# Autodesk Inventor assembly: Center Frame SEC
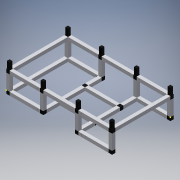
[picture p0: Inventor's stored thumbnail of the model, 180x180]
Saved by Autodesk Inventor 2017 (Build 210142000, 142)
## iProperties
Created: 2019-12-06
Part Number: Center Frame SEC
Document SubType Name: Assembly
Designer: S346553810
Author: S346553810
## Documents named in this file (7)
- \\ad.ocdsb.ca\studenthome\3\S338674153\FRC 2020\FullRobotRefactor\SubFrame\Center Frame SEC.iam
- \\ad.ocdsb.ca\studenthome\3\S338674153\FRC 2020\FullRobotRefactor\SubFrame\Center Assembly.iam
- \\ad.ocdsb.ca\studenthome\3\S338674153\FRC 2020\FullRobotRefactor\SubFrame\Frame End.iam
- \\ad.ocdsb.ca\studenthome\3\S338674153\FRC 2020\FullRobotRefactor\SubFrame\90 joint piece.ipt
- \\ad.ocdsb.ca\studenthome\3\S338674153\FRC 2020\FullRobotRefactor\SubFrame\lower piece.ipt
- \\ad.ocdsb.ca\studenthome\3\S338674153\FRC 2020\FullRobotRefactor\SubFrame\roller hole piece.ipt
- \\ad.ocdsb.ca\studenthome\3\S338674153\FRC 2020\FullRobotRefactor\SubFrame\Kipp K0619.ipt
## Components (12 placed, 6 different names)
1. Center Assembly:1 [sub-assembly] — Flush:33, Flush:34, Flush:35, Mate:36
2. Frame End:1 [sub-assembly] — Mate:29, Mate:30, Mate:31, Flush:26, Flush:27, Mate:34, Flush:28, Flush:29, Mate:35, Flush:30, Flush:32, Flush:33, Flush:34, Flush:35, Mate:36
3. Frame End:2 [sub-assembly] — Mate:33, Flush:22, Flush:23
4. 90 joint piece:1 — Mate:24, Flush:20, Flush:21
5. 90 joint piece:2 — Mate:23, Flush:18, Flush:19, Mate:33, Flush:22
6. lower piece:1 — Flush:24, Flush:25, Flush:31, Mate:37
7. roller hole piece:2 — Mate:23, Flush:18, Flush:19, Flush:23
8. roller hole piece:3 — Mate:24, Flush:20, Flush:21
9. roller hole piece:4 — Mate:29, Mate:30, Mate:31
10. roller hole piece:5 — Flush:28, Flush:29, Mate:35
11. Kipp K0619:1 — Flush:24, Flush:25, Flush:26, Flush:27, Mate:34, Mate:37
12. Kipp K0619:2 — Flush:30, Flush:31, Flush:32
## Relationships (28: Flush 18, Mate 10)
- Mate:23: 90 joint piece:2 ↔ roller hole piece:2
- Flush:18: 90 joint piece:2 ↔ roller hole piece:2
- Flush:19: 90 joint piece:2 ↔ roller hole piece:2
- Mate:24: 90 joint piece:1 ↔ roller hole piece:3
- Flush:20: 90 joint piece:1 ↔ roller hole piece:3
- Flush:21: 90 joint piece:1 ↔ roller hole piece:3
- Mate:29: Frame End:1 ↔ roller hole piece:4
- Mate:30: Frame End:1 ↔ roller hole piece:4
- Mate:31: Frame End:1 ↔ roller hole piece:4
- Mate:33: Frame End:2 ↔ 90 joint piece:2
- Flush:22: Frame End:2 ↔ 90 joint piece:2
- Flush:23: Frame End:2 ↔ roller hole piece:2
- Flush:24: lower piece:1 ↔ Kipp K0619:1
- Flush:25: lower piece:1 ↔ Kipp K0619:1
- Flush:26: Frame End:1 ↔ Kipp K0619:1
- Flush:27: Frame End:1 ↔ Kipp K0619:1
- Mate:34: Frame End:1 ↔ Kipp K0619:1
- Flush:28: Frame End:1 ↔ roller hole piece:5
- Flush:29: Frame End:1 ↔ roller hole piece:5
- Mate:35: Frame End:1 ↔ roller hole piece:5
- Flush:30: Frame End:1 ↔ Kipp K0619:2
- Flush:31: lower piece:1 ↔ Kipp K0619:2
- Flush:32: Frame End:1 ↔ Kipp K0619:2
- Flush:33: Center Assembly:1 ↔ Frame End:1
- Flush:34: Center Assembly:1 ↔ Frame End:1
- Flush:35: Center Assembly:1 ↔ Frame End:1
- Mate:36: Center Assembly:1 ↔ Frame End:1
- Mate:37: lower piece:1 ↔ Kipp K0619:1
